# Autodesk Inventor assembly: mould_top_p1
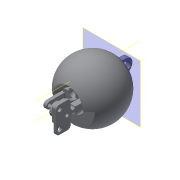
[picture p0: Inventor's stored thumbnail of the model, 180x180]
Saved by Autodesk Inventor 2017 (Build 210142000, 142)
## iProperties
Created: 2018-06-07
Part Number: mould_top_p1
Document SubType Name: Assembly
Designer: Nic
Author: Nic
## Documents named in this file (3)
- C:\Users\Nic\Documents\Antenna\mould_top_p1.iam
- C:\Users\Nic\Documents\Antenna\middle_segment_v2.ipt
- C:\Users\Nic\Documents\Antenna\sensor_pad.ipt
## Components (2 placed, 2 different names)
1. middle_segment_v2:1 — Mate:2, Flush:1, Angle:1
2. sensor_pad:1 — Mate:1, Flush:1, Angle:1
## Relationships (4: Mate 2, Flush 1, Angle 1)
- Mate:1: sensor_pad:1
- Mate:2: middle_segment_v2:1
- Flush:1 (1 mm): middle_segment_v2:1 ↔ sensor_pad:1
- Angle:1 (0 deg): middle_segment_v2:1 ↔ sensor_pad:1
